# Autodesk Inventor assembly: Lamp
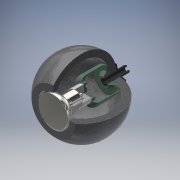
[picture p0: Inventor's stored thumbnail of the model, 180x180]
Saved by Autodesk Inventor 2018.2 (Build 222227000, 227)
## iProperties
Created: 2018-01-26
Part Number: Lamp
Material: Generisch
Document SubType Name: Assembly
Designer: JochenAlt
Author: JochenAlt
## Documents named in this file (8)
- D:\Projects\concretelamp\CAD\Lamp.iam
- D:\Projects\concretelamp\CAD\CableStrainRelief.ipt
- D:\Projects\concretelamp\CAD\Inlet.ipt
- D:\Projects\concretelamp\CAD\Lamp.ipt
- D:\Projects\concretelamp\CAD\Bulb GU10\Bulb GU10.iam
- D:\Projects\concretelamp\CAD\GU10-Socket.ipt
- C:\Users\JochenAlt\Documents\Inventor\Content Center Files\R2018\de-DE\DIN 912\DIN 912 - M3 x 0,5 x 16 x 14,75.ipt
- C:\Users\JochenAlt\Documents\Inventor\Content Center Files\R2018\de-DE\BS 3692(1)\BS 3692 - M3(1).ipt
## Components (9 placed, 7 different names)
1. Kabelzugentlastung:1 — Passend:1, Passend:2, Passend:3
2. V5 Inlet:1 — Passend:1, Passend:7, Passend:8, Passend:17, Passend:19
3. Lamp:1 — Passend:2, Passend:3
4. Bulb GU10:1 [sub-assembly] — Passend:9, Passend:10, Passend:11
5. GU10-Socket:1 — Passend:7, Passend:8, Passend:9, Passend:10, Passend:11, Passend:12, Passend:13, Passend:14, Passend:15
6. DIN 912 - ersetzt durch DIN EN ISO 4762 M3 x 16:1 — Passend:12, Passend:13, Passend:16
7. DIN 912 - ersetzt durch DIN EN ISO 4762 M3 x 16:2 — Passend:14, Passend:15, Passend:18
8. BS 3692 - Metrisch M3:1 — Passend:16, Passend:17
9. BS 3692 - Metrisch M3:2 — Passend:18, Passend:19
## Relationships (16: Mate 16)
- Passend:1 [Mate]: Kabelzugentlastung:1 ↔ V5 Inlet:1
- Passend:2 [Mate]: Kabelzugentlastung:1 ↔ Lamp:1
- Passend:3 [Mate] (0.5 mm): Kabelzugentlastung:1 ↔ Lamp:1
- Passend:7 [Mate]: V5 Inlet:1 ↔ GU10-Socket:1
- Passend:8 [Mate]: V5 Inlet:1 ↔ GU10-Socket:1
- Passend:9 [Mate]: Bulb GU10:1 ↔ GU10-Socket:1
- Passend:10 [Mate] (0.054 mm): Bulb GU10:1 ↔ GU10-Socket:1
- Passend:11 [Mate] (0.5 mm): Bulb GU10:1 ↔ GU10-Socket:1
- Passend:12 [Mate]: GU10-Socket:1 ↔ DIN 912 - ersetzt durch DIN EN ISO 4762 M3 x 16:1
- Passend:13 [Mate]: GU10-Socket:1 ↔ DIN 912 - ersetzt durch DIN EN ISO 4762 M3 x 16:1
- Passend:14 [Mate]: GU10-Socket:1 ↔ DIN 912 - ersetzt durch DIN EN ISO 4762 M3 x 16:2
- Passend:15 [Mate]: GU10-Socket:1 ↔ DIN 912 - ersetzt durch DIN EN ISO 4762 M3 x 16:2
- Passend:16 [Mate]: DIN 912 - ersetzt durch DIN EN ISO 4762 M3 x 16:1 ↔ BS 3692 - Metrisch M3:1
- Passend:17 [Mate]: V5 Inlet:1 ↔ BS 3692 - Metrisch M3:1
- Passend:18 [Mate]: DIN 912 - ersetzt durch DIN EN ISO 4762 M3 x 16:2 ↔ BS 3692 - Metrisch M3:2
- Passend:19 [Mate]: V5 Inlet:1 ↔ BS 3692 - Metrisch M3:2
